# Autodesk Inventor assembly: CycloidalTestAssembly
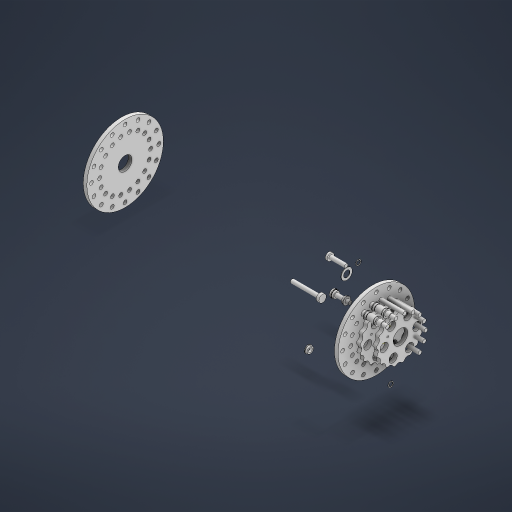
[picture p0: Inventor's stored thumbnail of the model, 512x512]
Saved by Autodesk Inventor 2024 (Build 280153000, 153)
## iProperties
Created: 2024-03-11
Part Number: CycloidalTestAssembly
Document SubType Name: Assembly
Designer: avsar
Author: avsar
## Documents named in this file (19)
- C:\Users\avsar\Documents\Inventor\RCR_Arm\Cycloidial Gearbox Example\CycloidalTestAssembly.iam
- C:\Users\avsar\Documents\Inventor\RCR_Arm\Cycloidial Gearbox Example\HousingFaceMount.ipt
- C:\Users\avsar\Documents\Inventor\RCR_Arm\Arm_V4\CycloidalGearBoxes\StageOneGearBox\Gearbox_MainBody.ipt
- C:\Users\avsar\Documents\Inventor\RCR_Arm\Cycloidial Gearbox Example\HousingExampleLid.ipt
- C:\Users\avsar\Documents\Inventor\RCR_Arm\Cycloidial Gearbox Example\BearingShaft.ipt
- C:\Users\avsar\Documents\Inventor\RCR_Arm\Arm_V4\CycloidalGearBoxes\StageOneGearBox\HousingInputFaceSpacer.ipt
- C:\Users\avsar\Documents\Inventor\RCR_Arm\Cycloidial Gearbox Example\FakeAssBearing.ipt
- C:\Users\avsar\Documents\Inventor\RCR_Arm\Arm_V4\CycloidalGearBoxes\StageOneGearBox\RollerBearingShaft.ipt
- C:\Users\avsar\Documents\Inventor\RCR_Arm\Arm_V4\CycloidalGearBoxes\StageOneGearBox\HousingLidSpacer.ipt
- C:\Users\avsar\Documents\Inventor\RCR_Arm\Cycloidial Gearbox Example\InputShaftFakeBearing.ipt
- C:\Users\avsar\Documents\Inventor\RCR_Arm\Arm_V4\CycloidalGearBoxes\StageOneGearBox\InputSpacer.ipt
- C:\Users\avsar\Documents\Inventor\RCR_Arm\Arm_V4\CycloidalGearBoxes\StageOneGearBox\EccentricBearingShaft.ipt
- C:\Users\avsar\Documents\Inventor\RCR_Arm\Cycloidial Gearbox Example\FakeButtonHead.ipt
- C:\Users\avsar\Documents\Inventor\RCR_Arm\Cycloidial Gearbox Example\NewCycloidalDisk.ipt
- C:\Users\avsar\Documents\Inventor\RCR_Arm\Arm_V4\CycloidalGearBoxes\StageOneGearBox\OutPutPlate.ipt
- C:\Users\avsar\Documents\Inventor\RCR_Arm\Arm_V4\CycloidalGearBoxes\StageOneGearBox\OutputPlateSpacer.ipt
- C:\Users\avsar\Documents\Inventor\RCR_Arm\Arm_V4\CycloidalGearBoxes\StageOneGearBox\OutputBearingDistanceRing.ipt
- C:\Users\avsar\Documents\Inventor\RCR_Arm\Cycloidial Gearbox Example\32mmFakeBearing.ipt
- C:\Users\avsar\Documents\Inventor\RCR_Arm\Cycloidial Gearbox Example\Flange.ipt
## Components (41 placed, 18 different names)
1. HousingFaceMount:1 — Mate:1, Mate:2, Mate:3, Mate:4, Mate:5, Mate:7, Mate:8, Mate:9, Mate:10, Mate:11, Mate:12, Mate:13, Mate:14, Mate:15, Mate:16, Mate:17, Mate:18, Mate:19, Mate:20, Mate:21, Mate:22, Mate:23, Mate:24, Mate:25, Mate:35, Mate:36, Mate:70
2. Gearbox_MainBody:1 — Mate:1, Mate:2, Mate:3, Mate:6
3. HousingExampleLid:1 — Mate:4, Mate:5, Mate:6, Mate:54, Mate:55
4. BearingShaft:1 — Mate:7, Mate:8, Mate:26, Mate:28, Mate:30, Mate:32
5. BearingShaft:3 — Mate:9, Mate:10, Mate:74
6. BearingShaft:4 — Mate:11, Mate:12
7. BearingShaft:5 — Mate:13, Mate:14
8. BearingShaft:6 — Mate:15, Mate:16
9. BearingShaft:7 — Mate:17, Mate:18
10. BearingShaft:8 — Mate:19, Mate:20
11. BearingShaft:9 — Mate:21, Mate:22
12. BearingShaft:10 — Mate:23, Mate:24
13. BearingShaft:11
14. HousingInputFaceSpacer:1 — Mate:25, Mate:26, Mate:27
15. FakeAssBearing:1 — Mate:27, Mate:28, Mate:29, Mate:75
16. RollerBearingShaft:1 — Mate:29, Mate:30, Mate:31, Mate:34, Tangent:1
17. FakeAssBearing:2 — Mate:31, Mate:32, Mate:33, Mate:44, Mate:76
18. HousingLidSpacer:1 — Mate:33, Mate:34
19. InputShaftFakeBearing:1 — Mate:35, Mate:36, Mate:37, Mate:38
20. InputSpacer:1 — Mate:37, Mate:38, Mate:39, Mate:40
21. EccentricBearingShaft:1 — Mate:39, Mate:40, Mate:43
22. NewCycloidalDisk:2 — Mate:43, Mate:44
23. OutPutPlate:1 — Mate:54, Mate:56
24. OutputBearingDistanceRing:1 — Mate:55, Mate:56, Mate:57, Mate:58
25. 32mmFakeBearing:1 — Mate:57, Mate:58
26. FakeAssBearing:6
27. OutputPlateSpacer:2
28. HousingInputFaceSpacer:2 — Mate:70, Mate:71, Mate:74
29. FakeAssBearing:7 — Mate:72
30. RollerBearingShaft:2 — Mate:71, Mate:72, Tangent:2
31. FakeAssBearing:8 — Mate:73
32. HousingLidSpacer:2 — Mate:73
33. FakeButtonHead:1
34. FakeAssBearing:9
35. FakeAssBearing:10
36. NewCycloidalDisk:3 — Mate:75, Tangent:1, Tangent:2
37. Flange:1
38. OutputPlateSpacer:3
39. HousingFaceMount:2
40. FakeButtonHead:2
41. NewCycloidalDisk:4 — Mate:76
## Relationships (61: Mate 59, Tangent 2)
- Mate:1: HousingFaceMount:1 ↔ Gearbox_MainBody:1
- Mate:2: HousingFaceMount:1 ↔ Gearbox_MainBody:1
- Mate:3: HousingFaceMount:1 ↔ Gearbox_MainBody:1
- Mate:4: HousingFaceMount:1 ↔ HousingExampleLid:1
- Mate:5: HousingFaceMount:1 ↔ HousingExampleLid:1
- Mate:6: Gearbox_MainBody:1 ↔ HousingExampleLid:1
- Mate:7: HousingFaceMount:1 ↔ BearingShaft:1
- Mate:8: HousingFaceMount:1 ↔ BearingShaft:1
- Mate:9: HousingFaceMount:1 ↔ BearingShaft:3
- Mate:10: HousingFaceMount:1 ↔ BearingShaft:3
- Mate:11: HousingFaceMount:1 ↔ BearingShaft:4
- Mate:12: HousingFaceMount:1 ↔ BearingShaft:4
- Mate:13: HousingFaceMount:1 ↔ BearingShaft:5
- Mate:14: HousingFaceMount:1 ↔ BearingShaft:5
- Mate:15: HousingFaceMount:1 ↔ BearingShaft:6
- Mate:16: HousingFaceMount:1 ↔ BearingShaft:6
- Mate:17: HousingFaceMount:1 ↔ BearingShaft:7
- Mate:18: HousingFaceMount:1 ↔ BearingShaft:7
- Mate:19: HousingFaceMount:1 ↔ BearingShaft:8
- Mate:20: HousingFaceMount:1 ↔ BearingShaft:8
- Mate:21: HousingFaceMount:1 ↔ BearingShaft:9
- Mate:22: HousingFaceMount:1 ↔ BearingShaft:9
- Mate:23: HousingFaceMount:1 ↔ BearingShaft:10
- Mate:24: HousingFaceMount:1 ↔ BearingShaft:10
- Mate:25: HousingFaceMount:1 ↔ HousingInputFaceSpacer:1
- Mate:26: BearingShaft:1 ↔ HousingInputFaceSpacer:1
- Mate:27: HousingInputFaceSpacer:1 ↔ FakeAssBearing:1
- Mate:28: BearingShaft:1 ↔ FakeAssBearing:1
- Mate:29: FakeAssBearing:1 ↔ RollerBearingShaft:1
- Mate:30: BearingShaft:1 ↔ RollerBearingShaft:1
- Mate:31: RollerBearingShaft:1 ↔ FakeAssBearing:2
- Mate:32: BearingShaft:1 ↔ FakeAssBearing:2
- Mate:33: FakeAssBearing:2 ↔ HousingLidSpacer:1
- Mate:34: RollerBearingShaft:1 ↔ HousingLidSpacer:1
- Mate:35: HousingFaceMount:1 ↔ InputShaftFakeBearing:1
- Mate:36: HousingFaceMount:1 ↔ InputShaftFakeBearing:1
- Mate:37: InputShaftFakeBearing:1 ↔ InputSpacer:1
- Mate:38: InputShaftFakeBearing:1 ↔ InputSpacer:1
- Mate:39: InputSpacer:1 ↔ EccentricBearingShaft:1
- Mate:40: InputSpacer:1 ↔ EccentricBearingShaft:1
- Mate:43: EccentricBearingShaft:1 ↔ NewCycloidalDisk:2
- Mate:44: FakeAssBearing:2 ↔ NewCycloidalDisk:2
- Mate:54: HousingExampleLid:1 ↔ OutPutPlate:1
- Mate:55: HousingExampleLid:1 ↔ OutputBearingDistanceRing:1
- Mate:56: OutPutPlate:1 ↔ OutputBearingDistanceRing:1
- Mate:57: OutputBearingDistanceRing:1 ↔ 32mmFakeBearing:1
- Mate:58: OutputBearingDistanceRing:1 ↔ 32mmFakeBearing:1
- [Mate]: HousingInputFaceSpacer:2 ↔ FakeAssBearing:7
- [Mate]: FakeAssBearing:7 ↔ RollerBearingShaft:2
- [Mate]: RollerBearingShaft:2 ↔ FakeAssBearing:8
- [Mate]: FakeAssBearing:8 ↔ HousingLidSpacer:2
- [Mate]: RollerBearingShaft:2 ↔ HousingLidSpacer:2
- Mate:70: HousingFaceMount:1 ↔ HousingInputFaceSpacer:2
- Mate:71: HousingInputFaceSpacer:2 ↔ RollerBearingShaft:2
- Mate:72: FakeAssBearing:7 ↔ RollerBearingShaft:2
- Mate:73: FakeAssBearing:8 ↔ HousingLidSpacer:2
- Mate:74: BearingShaft:3 ↔ HousingInputFaceSpacer:2
- Mate:75: FakeAssBearing:1 ↔ NewCycloidalDisk:3
- Tangent:1: RollerBearingShaft:1 ↔ NewCycloidalDisk:3
- Tangent:2: RollerBearingShaft:2 ↔ NewCycloidalDisk:3
- Mate:76: FakeAssBearing:2 ↔ NewCycloidalDisk:4
## Named parameters: d84_d36 = 0 mm, d85_d38 = 0 mm, d86_d40 = 0 mm, d87_d42 = 0 mm, d88_d43 = 0 mm
